# Autodesk Inventor assembly: window frame
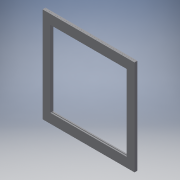
[picture p0: Inventor's stored thumbnail of the model, 180x180]
Saved by Autodesk Inventor 2017 (Build 210142000, 142)
## iProperties
Created: 2019-05-07
Part Number: window frame
Document SubType Name: Assembly
Designer: Roman
Author: Roman
## Documents named in this file (3)
- C:\Users\Roman\Documents\CAD\tegu rev2\upper walls\window wall\window rev2\window frame.iam
- C:\Users\Roman\Documents\CAD\tegu rev2\upper walls\window wall\window rev2\window outer.ipt
- C:\Users\Roman\Documents\CAD\tegu rev2\upper walls\window wall\window rev2\window inner.ipt
## Components (3 placed, 2 different names)
1. window outer:1 — Mate:1, Flush:1, Flush:2
2. window inner:1 — Mate:1, Flush:1, Flush:2, Mate:2, Flush:3, Flush:4
3. window outer:2 — Mate:2, Flush:3, Flush:4
## Relationships (6: Flush 4, Mate 2)
- Mate:1: window outer:1 ↔ window inner:1
- Flush:1: window outer:1 ↔ window inner:1
- Flush:2: window outer:1 ↔ window inner:1
- Mate:2: window inner:1 ↔ window outer:2
- Flush:3: window inner:1 ↔ window outer:2
- Flush:4: window inner:1 ↔ window outer:2
